# Autodesk Inventor assembly: Robot_face
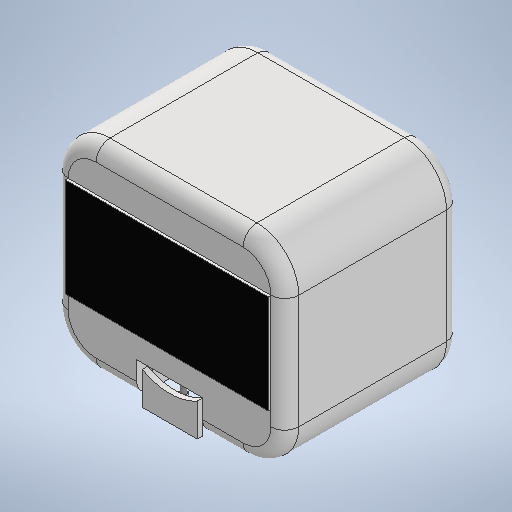
[picture p0: Inventor's stored thumbnail of the model, 512x512]
Saved by Autodesk Inventor 2025 (Build 290162010, 162A)
## iProperties
Created: 2024-07-17
Part Number: Robot_face
Document SubType Name: Assembly
Designer: saees
Author: saees
## Documents named in this file (3)
- C:\Users\saees\OneDrive\Documents\Inventor\Robot_face.iam
- C:\Users\saees\OneDrive\Documents\Inventor\Robot_face.ipt
- C:\Users\saees\OneDrive\Documents\Inventor\Robot_mouth.ipt
## Components (2 placed, 2 different names)
1. Robot_face:1 — Mate:1
2. Robot_mouth:1 — Mate:1
## Relationships (1: Mate 1)
- Mate:1: Robot_face:1 ↔ Robot_mouth:1
